# Autodesk Inventor assembly: HeadSlider
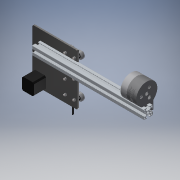
[picture p0: Inventor's stored thumbnail of the model, 180x180]
Saved by Autodesk Inventor 2017 (Build 210142000, 142)
## iProperties
Created: 2016-12-13
Part Number: HeadSlider
Document SubType Name: Assembly
Designer: umr
Mass: 1451.96 g
Surface Area: 2251.36 cm^2
Volume: 395.039 cm^3
Density: 3.67548 g/cm^3
Author: umr
## Documents named in this file (10)
- D:\SeniorProject\Models2\Head\HeadSlider.iam
- D:\SeniorProject\Models2\Head\HeadPlate.ipt
- D:\SeniorProject\Models2\Head\Solid Wheel with Eccentric Spacer Assembly.iam
- D:\SeniorProject\Models2\Head\Motor.ipt
- D:\SeniorProject\Models2\Head\GT2 20 Tooth Pulley.ipt
- D:\SeniorProject\Models2\Head\HeaderSliderBelt.ipt
- D:\SeniorProject\Models2\Head\HeaderFixer.ipt
- D:\SeniorProject\Models2\Head\M5 Screw with Tee Nut.iam
- D:\SeniorProject\Models2\Head\UTM Cover.ipt
- D:\SeniorProject\Models2\Head\UTM.ipt
## Components (20 placed, 9 different names)
1. HeadPlate:1 — Mate:1, Mate:2, Mate:3, Mate:4, Mate:5, Mate:6, Mate:7, Mate:8, Mate:9, Mate:10, Mate:11, Mate:12, Mate:13, Mate:14, Mate:15, Mate:16, Mate:17, Mate:18, Mate:20, Mate:21, Mate:22, Mate:23, Mate:24
2. Solid Wheel with Eccentric Spacer Assembly:1 [sub-assembly] — Mate:3, Mate:8
3. Solid Wheel with Eccentric Spacer Assembly:2 [sub-assembly] — Mate:4, Mate:9, Tangent:1
4. Solid Wheel with Eccentric Spacer Assembly:3 [sub-assembly] — Mate:6, Mate:11
5. Solid Wheel with Eccentric Spacer Assembly:4 [sub-assembly] — Mate:1, Mate:13
6. Solid Wheel with Eccentric Spacer Assembly:5 [sub-assembly] — Mate:2, Mate:14
7. Solid Wheel with Eccentric Spacer Assembly:6 [sub-assembly] — Mate:5, Mate:12
8. Solid Wheel with Eccentric Spacer Assembly:7 [sub-assembly] — Mate:7, Mate:10, Tangent:2
9. Motor:1 — Mate:15, Mate:16, Mate:17, Mate:18, Mate:19
10. GT2 20 Tooth Pulley:1 — Mate:19, Mate:20
11. HeaderSliderBelt:1 — Tangent:1, Tangent:2
12. HeaderFixer:1 — Mate:25, Mate:26, Mate:27, Mate:28, Mate:29, Mate:30, Mate:31, Mate:33, Mate:34, Mate:35, Mate:36, Mate:41
13. M5 Screw with Tee Nut:1 [sub-assembly] — Mate:21, Mate:23, Mate:25, Mate:26
14. M5 Screw with Tee Nut:2 [sub-assembly] — Mate:22, Mate:24, Mate:27
15. UTM Cover:1 — Mate:32, Flush:1, Flush:2, Mate:39, Mate:40
16. UTM:1 — Mate:32, Flush:1, Flush:2, Mate:37, Mate:38, Mate:41
17. M5 Screw with Tee Nut:3 [sub-assembly] — Mate:28, Mate:34, Mate:39
18. M5 Screw with Tee Nut:4 [sub-assembly] — Mate:29, Mate:33, Mate:38
19. M5 Screw with Tee Nut:5 [sub-assembly] — Mate:31, Mate:36, Mate:37
20. M5 Screw with Tee Nut:6 [sub-assembly] — Mate:30, Mate:35, Mate:40
## Relationships (45: Mate 41, Tangent 2, Flush 2)
- Mate:1: HeadPlate:1 ↔ Solid Wheel with Eccentric Spacer Assembly:4
- Mate:2: HeadPlate:1 ↔ Solid Wheel with Eccentric Spacer Assembly:5
- Mate:3: HeadPlate:1 ↔ Solid Wheel with Eccentric Spacer Assembly:1
- Mate:4: HeadPlate:1 ↔ Solid Wheel with Eccentric Spacer Assembly:2
- Mate:5: HeadPlate:1 ↔ Solid Wheel with Eccentric Spacer Assembly:6
- Mate:6: HeadPlate:1 ↔ Solid Wheel with Eccentric Spacer Assembly:3
- Mate:7: HeadPlate:1 ↔ Solid Wheel with Eccentric Spacer Assembly:7
- Mate:8: HeadPlate:1 ↔ Solid Wheel with Eccentric Spacer Assembly:1
- Mate:9: HeadPlate:1 ↔ Solid Wheel with Eccentric Spacer Assembly:2
- Mate:10: HeadPlate:1 ↔ Solid Wheel with Eccentric Spacer Assembly:7
- Mate:11: HeadPlate:1 ↔ Solid Wheel with Eccentric Spacer Assembly:3
- Mate:12: HeadPlate:1 ↔ Solid Wheel with Eccentric Spacer Assembly:6
- Mate:13: HeadPlate:1 ↔ Solid Wheel with Eccentric Spacer Assembly:4
- Mate:14: HeadPlate:1 ↔ Solid Wheel with Eccentric Spacer Assembly:5
- Mate:15: HeadPlate:1 ↔ Motor:1
- Mate:16: HeadPlate:1 ↔ Motor:1
- Mate:17: HeadPlate:1 ↔ Motor:1
- Mate:18: HeadPlate:1 ↔ Motor:1
- Mate:19: Motor:1 ↔ GT2 20 Tooth Pulley:1
- Mate:20: HeadPlate:1 ↔ GT2 20 Tooth Pulley:1
- Tangent:1: Solid Wheel with Eccentric Spacer Assembly:2 ↔ HeaderSliderBelt:1
- Tangent:2: Solid Wheel with Eccentric Spacer Assembly:7 ↔ HeaderSliderBelt:1
- Mate:21: HeadPlate:1 ↔ M5 Screw with Tee Nut:1
- Mate:22: HeadPlate:1 ↔ M5 Screw with Tee Nut:2
- Mate:23: HeadPlate:1 ↔ M5 Screw with Tee Nut:1
- Mate:24: HeadPlate:1 ↔ M5 Screw with Tee Nut:2
- Mate:25 (1 mm): HeaderFixer:1 ↔ M5 Screw with Tee Nut:1
- Mate:26 (3.5 mm): HeaderFixer:1 ↔ M5 Screw with Tee Nut:1
- Mate:27 (3.5 mm): HeaderFixer:1 ↔ M5 Screw with Tee Nut:2
- Mate:28 (1 mm): HeaderFixer:1 ↔ M5 Screw with Tee Nut:3
- Mate:29 (1 mm): HeaderFixer:1 ↔ M5 Screw with Tee Nut:4
- Mate:30 (1 mm): HeaderFixer:1 ↔ M5 Screw with Tee Nut:6
- Mate:31 (1 mm): HeaderFixer:1 ↔ M5 Screw with Tee Nut:5
- Mate:32: UTM Cover:1 ↔ UTM:1
- Flush:1: UTM Cover:1 ↔ UTM:1
- Flush:2: UTM Cover:1 ↔ UTM:1
- Mate:33 (3.5 mm): HeaderFixer:1 ↔ M5 Screw with Tee Nut:4
- Mate:34 (3.5 mm): HeaderFixer:1 ↔ M5 Screw with Tee Nut:3
- Mate:35 (3.5 mm): HeaderFixer:1 ↔ M5 Screw with Tee Nut:6
- Mate:36 (3.5 mm): HeaderFixer:1 ↔ M5 Screw with Tee Nut:5
- Mate:37: UTM:1 ↔ M5 Screw with Tee Nut:5
- Mate:38: UTM:1 ↔ M5 Screw with Tee Nut:4
- Mate:39: UTM Cover:1 ↔ M5 Screw with Tee Nut:3
- Mate:40: UTM Cover:1 ↔ M5 Screw with Tee Nut:6
- Mate:41: HeaderFixer:1 ↔ UTM:1
